# Autodesk Inventor assembly: end door assembly.ipt
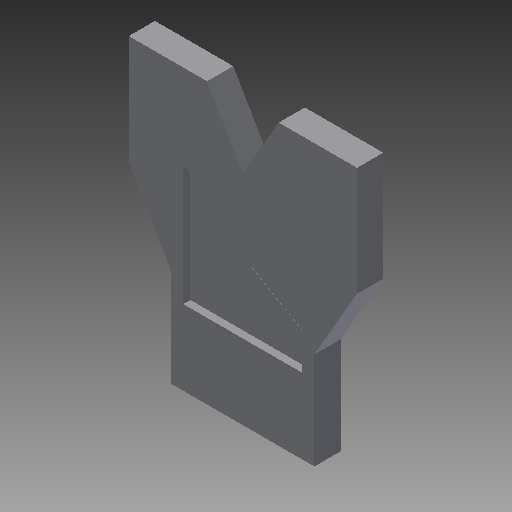
[picture p0: Inventor's stored thumbnail of the model, 512x512]
Saved by Autodesk Inventor 2017 (Build 210142000, 142)
## iProperties
Created: 2018-03-10
Part Number: end door assembly.ipt
Document SubType Name: Assembly
Designer: Braxton
Author: Braxton
## Documents named in this file (7)
- D:\School\Game develpment\geoscape\doors\end door\assembly\end door assembly.ipt.iam
- D:\School\Game develpment\geoscape\doors\end door\end door frame.ipt
- D:\School\Game develpment\geoscape\doors\end door\bottom door.ipt
- D:\School\Game develpment\geoscape\doors\end door\top left door.ipt
- D:\School\Game develpment\geoscape\doors\end door\top right door.ipt
- D:\School\Game develpment\geoscape\doors\end door\bottom and top hiding bar.ipt
- D:\School\Game develpment\geoscape\doors\end door\left and right hiding bar.ipt
## Components (12 placed, 12 different names)
1. end door frame:1 — Mate:10, Mate:11, Mate:12, Mate:13, Mate:14, Mate:15, Mate:16, Mate:17, Mate:18, Mate:19, Mate:20, Mate:21, Mate:22, Mate:23, Mate:24, Mate:25, Mate:26, Mate:27, Mate:28, Mate:29, Mate:30, Mate:31, Mate:32, Mate:33, Mate:34, Mate:35, Mate:36, Mate:37, Mate:38, Mate:39, Mate:40, Mate:41
2. bottom door:1 — Mate:34, Mate:35, Mate:42
3. top right door:1 — Mate:39, Mate:40, Mate:41, Flush:1
4. top left door:1 — Mate:36, Mate:37, Mate:38, Flush:1, Mate:42
5. front top hiding bar — Mate:10, Mate:11, Mate:12
6. front bottom hiding bar — Mate:25, Mate:26, Mate:27
7. front right hiding bar — Mate:28, Mate:29, Mate:30
8. front left hiding bar — Mate:31, Mate:32, Mate:33
9. back bottom hiding bar — Mate:16, Mate:17, Mate:18
10. back top hiding bar — Mate:13, Mate:14, Mate:15
11. back right hiding bar — Mate:22, Mate:23, Mate:24
12. back left hiding bar — Mate:19, Mate:20, Mate:21
## Relationships (34: Mate 33, Flush 1)
- Mate:10: end door frame:1 ↔ front top hiding bar
- Mate:11: end door frame:1 ↔ front top hiding bar
- Mate:12: end door frame:1 ↔ front top hiding bar
- Mate:13: end door frame:1 ↔ back top hiding bar
- Mate:14: end door frame:1 ↔ back top hiding bar
- Mate:15: end door frame:1 ↔ back top hiding bar
- Mate:16: end door frame:1 ↔ back bottom hiding bar
- Mate:17: end door frame:1 ↔ back bottom hiding bar
- Mate:18: end door frame:1 ↔ back bottom hiding bar
- Mate:19: end door frame:1 ↔ back left hiding bar
- Mate:20: end door frame:1 ↔ back left hiding bar
- Mate:21: end door frame:1 ↔ back left hiding bar
- Mate:22: end door frame:1 ↔ back right hiding bar
- Mate:23: end door frame:1 ↔ back right hiding bar
- Mate:24: end door frame:1 ↔ back right hiding bar
- Mate:25: end door frame:1 ↔ front bottom hiding bar
- Mate:26: end door frame:1 ↔ front bottom hiding bar
- Mate:27: end door frame:1 ↔ front bottom hiding bar
- Mate:28: end door frame:1 ↔ front right hiding bar
- Mate:29: end door frame:1 ↔ front right hiding bar
- Mate:30: end door frame:1 ↔ front right hiding bar
- Mate:31: end door frame:1 ↔ front left hiding bar
- Mate:32: end door frame:1 ↔ front left hiding bar
- Mate:33: end door frame:1 ↔ front left hiding bar
- Mate:34: end door frame:1 ↔ bottom door:1
- Mate:35: end door frame:1 ↔ bottom door:1
- Mate:36: end door frame:1 ↔ top left door:1
- Mate:37: end door frame:1 ↔ top left door:1
- Mate:38: end door frame:1 ↔ top left door:1
- Mate:39: end door frame:1 ↔ top right door:1
- Mate:40: end door frame:1 ↔ top right door:1
- Mate:41: end door frame:1 ↔ top right door:1
- Flush:1: top right door:1 ↔ top left door:1
- Mate:42: bottom door:1 ↔ top left door:1
